# Autodesk Inventor assembly: BODY
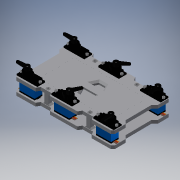
[picture p0: Inventor's stored thumbnail of the model, 180x180]
Saved by Autodesk Inventor 2017.3 (Build 213256000, 256)
## iProperties
Created: 2017-09-24
Part Number: BODY
Document SubType Name: Assembly
Designer: Alexander Miller
Author: Alexander Miller
## Documents named in this file (10)
- X:\Alex\Documents\Git\HeRo-Mini\Hardware\BODY.iam
- X:\Alex\Documents\Git\HeRo-Mini\Hardware\BODY_BOTTOM.ipt
- X:\Alex\Documents\Git\HeRo-Mini\Hardware\BODY_TOP.ipt
- X:\Alex\Documents\Git\HeRo-Mini\Hardware\SERVO.iam
- X:\Alex\Documents\Git\HeRo-Mini\Hardware\BODY_TOP_COVER.ipt
- X:\Alex\Documents\Git\HeRo-Mini\Hardware\MAGNET.ipt
- X:\Alex\Documents\Git\HeRo-Mini\Hardware\NUT_3MM.ipt
- X:\Alex\Documents\Git\HeRo-Mini\Hardware\M3_SCREW_20MM.ipt
- X:\Alex\Documents\Git\HeRo-Mini\Hardware\NUT_2MM.ipt
- X:\Alex\Documents\Git\HeRo-Mini\Hardware\M2_SCREW_8MM.ipt
## Components (59 placed, 9 different names)
1. BODY_BOTTOM:1 — Rigid:8, Rigid:9, Rigid:10, Rigid:11, Rigid:12, Rigid:13, Rigid:22, Rigid:23, Rigid:24, Rigid:25, Rigid:26, Rigid:27, Rigid:28, Rigid:29, Rigid:34, Rigid:35, Rigid:36, Rigid:37, Rigid:38, Rigid:39
2. BODY_TOP:1 — Rigid:7, Rigid:30, Rigid:31, Rigid:32, Rigid:33, Rigid:40, Rigid:41, Rigid:42, Rigid:43, Rigid:44, Rigid:45, Rigid:46, Rigid:47, Rigid:48, Rigid:49, Rigid:50, Rigid:51, Rigid:63, Rigid:64, Rigid:65, Rigid:66, Cylindrical:68
3. SERVO:1 [sub-assembly] — Rigid:7, Rigid:13, Rigid:52, Rigid:53
4. SERVO:2 [sub-assembly] — Rigid:12, Rotational:1, Rigid:54
5. SERVO:3 [sub-assembly] — Rigid:11, Rigid:55, Rigid:56
6. SERVO:4 [sub-assembly] — Rigid:10, Rigid:57, Rigid:58
7. SERVO:5 [sub-assembly] — Rigid:9, Rigid:59, Rigid:60
8. SERVO:6 [sub-assembly] — Rigid:8, Rigid:61, Rigid:62
9. BODY_TOP_COVER:1 — Rigid:18, Rigid:19, Rigid:20, Rigid:21
10. MAGNET:1 — Rigid:64
11. MAGNET:2 — Rigid:63
12. MAGNET:3 — Rigid:66
13. MAGNET:4 — Rigid:18, Cylindrical:68
14. MAGNET:5 — Rigid:65
15. MAGNET:6 — Rigid:20
16. MAGNET:7 — Rigid:21
17. MAGNET:8 — Rigid:19
18. NUT_3MM:1 — Rigid:22
19. NUT_3MM:2 — Rigid:24
20. NUT_3MM:3 — Rigid:26
21. NUT_3MM:4 — Rigid:23
22. NUT_3MM:5 — Rigid:27
23. NUT_3MM:6 — Rigid:25
24. NUT_3MM:7 — Rigid:29
25. NUT_3MM:8 — Rigid:28
26. M3_SCREW_20MM:1 — Rigid:30
27. M3_SCREW_20MM:2 — Rigid:31
28. M3_SCREW_20MM:3 — Rigid:32
29. M3_SCREW_20MM:4 — Rigid:33
30. NUT_3MM:9 — Rigid:35
31. NUT_3MM:10 — Rigid:34
32. NUT_3MM:11 — Rigid:36
33. NUT_3MM:12 — Rigid:37
34. NUT_3MM:13 — Rigid:39
35. NUT_3MM:14 — Rigid:38
36. NUT_2MM:1 — Rigid:40
37. NUT_2MM:2 — Rigid:44
38. NUT_2MM:3 — Rigid:46
39. NUT_2MM:4 — Rigid:47
40. NUT_2MM:5 — Rigid:50
41. NUT_2MM:6 — Rigid:51
42. NUT_2MM:7 — Rigid:41
43. NUT_2MM:8 — Rigid:42
44. NUT_2MM:9 — Rigid:43
45. NUT_2MM:10 — Rigid:45
46. NUT_2MM:11 — Rigid:49
47. NUT_2MM:12 — Rigid:48
48. M2_SCREW_8MM:1 — Rigid:52
49. M2_SCREW_8MM:2 — Rigid:53
50. M2_SCREW_8MM:3 — Rotational:1
51. M2_SCREW_8MM:4 — Rigid:54
52. M2_SCREW_8MM:5 — Rigid:55
53. M2_SCREW_8MM:6 — Rigid:56
54. M2_SCREW_8MM:7 — Rigid:57
55. M2_SCREW_8MM:8 — Rigid:58
56. M2_SCREW_8MM:9 — Rigid:59
57. M2_SCREW_8MM:10 — Rigid:60
58. M2_SCREW_8MM:11 — Rigid:61
59. M2_SCREW_8MM:12 — Rigid:62
## Relationships (58: WeldJoint 56, RevoluteJoint 1, CylindricalJoint 1)
- Rigid:7 [WeldJoint]: BODY_TOP:1 ↔ SERVO:1
- Rigid:8 [WeldJoint]: BODY_BOTTOM:1 ↔ SERVO:6
- Rigid:9 [WeldJoint]: BODY_BOTTOM:1 ↔ SERVO:5
- Rigid:10 [WeldJoint]: BODY_BOTTOM:1 ↔ SERVO:4
- Rigid:11 [WeldJoint]: BODY_BOTTOM:1 ↔ SERVO:3
- Rigid:12 [WeldJoint]: BODY_BOTTOM:1 ↔ SERVO:2
- Rigid:13 [WeldJoint]: BODY_BOTTOM:1 ↔ SERVO:1
- Rigid:18 [WeldJoint]: BODY_TOP_COVER:1 ↔ MAGNET:4
- Rigid:19 [WeldJoint]: BODY_TOP_COVER:1 ↔ MAGNET:8
- Rigid:20 [WeldJoint]: BODY_TOP_COVER:1 ↔ MAGNET:6
- Rigid:21 [WeldJoint]: BODY_TOP_COVER:1 ↔ MAGNET:7
- Rigid:22 [WeldJoint]: BODY_BOTTOM:1 ↔ NUT_3MM:1
- Rigid:23 [WeldJoint]: BODY_BOTTOM:1 ↔ NUT_3MM:4
- Rigid:24 [WeldJoint]: BODY_BOTTOM:1 ↔ NUT_3MM:2
- Rigid:25 [WeldJoint]: BODY_BOTTOM:1 ↔ NUT_3MM:6
- Rigid:26 [WeldJoint]: BODY_BOTTOM:1 ↔ NUT_3MM:3
- Rigid:27 [WeldJoint]: BODY_BOTTOM:1 ↔ NUT_3MM:5
- Rigid:28 [WeldJoint]: BODY_BOTTOM:1 ↔ NUT_3MM:8
- Rigid:29 [WeldJoint]: BODY_BOTTOM:1 ↔ NUT_3MM:7
- Rigid:30 [WeldJoint]: BODY_TOP:1 ↔ M3_SCREW_20MM:1
- Rigid:31 [WeldJoint]: BODY_TOP:1 ↔ M3_SCREW_20MM:2
- Rigid:32 [WeldJoint]: BODY_TOP:1 ↔ M3_SCREW_20MM:3
- Rigid:33 [WeldJoint]: BODY_TOP:1 ↔ M3_SCREW_20MM:4
- Rigid:34 [WeldJoint]: BODY_BOTTOM:1 ↔ NUT_3MM:10
- Rigid:35 [WeldJoint]: BODY_BOTTOM:1 ↔ NUT_3MM:9
- Rigid:36 [WeldJoint]: BODY_BOTTOM:1 ↔ NUT_3MM:11
- Rigid:37 [WeldJoint]: BODY_BOTTOM:1 ↔ NUT_3MM:12
- Rigid:38 [WeldJoint]: BODY_BOTTOM:1 ↔ NUT_3MM:14
- Rigid:39 [WeldJoint]: BODY_BOTTOM:1 ↔ NUT_3MM:13
- Rigid:40 [WeldJoint]: BODY_TOP:1 ↔ NUT_2MM:1
- Rigid:41 [WeldJoint]: BODY_TOP:1 ↔ NUT_2MM:7
- Rigid:42 [WeldJoint]: BODY_TOP:1 ↔ NUT_2MM:8
- Rigid:43 [WeldJoint]: BODY_TOP:1 ↔ NUT_2MM:9
- Rigid:44 [WeldJoint]: BODY_TOP:1 ↔ NUT_2MM:2
- Rigid:45 [WeldJoint]: BODY_TOP:1 ↔ NUT_2MM:10
- Rigid:46 [WeldJoint]: BODY_TOP:1 ↔ NUT_2MM:3
- Rigid:47 [WeldJoint]: BODY_TOP:1 ↔ NUT_2MM:4
- Rigid:48 [WeldJoint]: BODY_TOP:1 ↔ NUT_2MM:12
- Rigid:49 [WeldJoint]: BODY_TOP:1 ↔ NUT_2MM:11
- Rigid:50 [WeldJoint]: BODY_TOP:1 ↔ NUT_2MM:5
- Rigid:51 [WeldJoint]: BODY_TOP:1 ↔ NUT_2MM:6
- Rigid:52 [WeldJoint]: SERVO:1 ↔ M2_SCREW_8MM:1
- Rigid:53 [WeldJoint]: SERVO:1 ↔ M2_SCREW_8MM:2
- Rotational:1 [RevoluteJoint]: SERVO:2 ↔ M2_SCREW_8MM:3
- Rigid:54 [WeldJoint]: SERVO:2 ↔ M2_SCREW_8MM:4
- Rigid:55 [WeldJoint]: SERVO:3 ↔ M2_SCREW_8MM:5
- Rigid:56 [WeldJoint]: SERVO:3 ↔ M2_SCREW_8MM:6
- Rigid:57 [WeldJoint]: SERVO:4 ↔ M2_SCREW_8MM:7
- Rigid:58 [WeldJoint]: SERVO:4 ↔ M2_SCREW_8MM:8
- Rigid:59 [WeldJoint]: SERVO:5 ↔ M2_SCREW_8MM:9
- Rigid:60 [WeldJoint]: SERVO:5 ↔ M2_SCREW_8MM:10
- Rigid:61 [WeldJoint]: SERVO:6 ↔ M2_SCREW_8MM:11
- Rigid:62 [WeldJoint]: SERVO:6 ↔ M2_SCREW_8MM:12
- Rigid:63 [WeldJoint]: BODY_TOP:1 ↔ MAGNET:2
- Rigid:64 [WeldJoint]: BODY_TOP:1 ↔ MAGNET:1
- Rigid:65 [WeldJoint]: BODY_TOP:1 ↔ MAGNET:5
- Rigid:66 [WeldJoint]: BODY_TOP:1 ↔ MAGNET:3
- Cylindrical:68: BODY_TOP:1 ↔ MAGNET:4
